# Autodesk Inventor assembly: RightSidePanelForCar
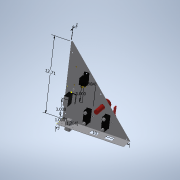
[picture p0: Inventor's stored thumbnail of the model, 180x180]
Saved by Autodesk Inventor 2021 (Build 250183000, 183)
## iProperties
Created: 2020-09-29
Part Number: RightSidePanelForCar
Document SubType Name: Assembly
Designer: Jonathan
Author: Jonathan
## Documents named in this file (9)
- D:\Scool\ECE 491\FullCarV2.2-20201122T225417Z-001\FullCarV2.2\SidePanels\RightSidePanelForCar.iam
- D:\Scool\ECE 491\Side_panels_11_1\RightSidePanel2020.ipt
- D:\Scool\ECE 491\FullCarV2.2-20201122T225417Z-001\FullCarV2.2\SidePanels\estop.ipt
- D:\Scool\ECE 491\FullCarV2.2-20201122T225417Z-001\FullCarV2.2\SidePanels\imdreset.ipt
- D:\Scool\ECE 491\FullCarV2.2-20201122T225417Z-001\FullCarV2.2\SidePanels\SSOK.ipt
- D:\Scool\ECE 491\FullCarV2.2-20201122T225417Z-001\FullCarV2.2\SidePanels\MRESET.iam
- D:\Scool\ECE 491\FullCarV2.2-20201122T225417Z-001\FullCarV2.2\SidePanels\DT_Flange_1.ipt
- D:\Scool\ECE 491\bosch-automotive-relay-0332209150-1.snapshot.3\Bosch 0 332 209 150.ipt
- D:\Scool\ECE 491\FullCarV2.2-20201122T225417Z-001\FullCarV2.2\SidePanels\9600K130_SBR RUBBER PUSH-IN GROMMET.ipt
## Components (9 placed, 8 different names)
1. RightSidePanel2020:1 — Mate:1, Mate:2, Mate:3, Mate:4, Mate:5, Mate:6, Mate:7, Mate:8, Mate:9, Mate:10, Mate:11, Mate:12, Mate:13, Insert:1, Mate:15, Mate:16
2. estop:1 — Mate:1, Mate:2
3. imdreset:1 — Mate:5, Mate:13
4. SSOK:1 — Mate:3, Mate:4, Mate:12
5. MRESET:1 [sub-assembly] — Mate:9, Mate:10, Mate:11
6. MRESET:2 [sub-assembly] — Mate:6, Mate:7, Mate:8
7. DT_Flange_1:1 — Mate:15
8. Bosch 0 332 209 150:1 — Mate:16
9. 9600K130_SBR RUBBER PUSH-IN GROMMET:1 — Insert:1
## Relationships (16: Mate 15, Insert 1)
- Mate:1: RightSidePanel2020:1 ↔ estop:1
- Mate:2: RightSidePanel2020:1 ↔ estop:1
- Mate:3: RightSidePanel2020:1 ↔ SSOK:1
- Mate:4: RightSidePanel2020:1 ↔ SSOK:1
- Mate:5: RightSidePanel2020:1 ↔ imdreset:1
- Mate:6: RightSidePanel2020:1 ↔ MRESET:2
- Mate:7: RightSidePanel2020:1 ↔ MRESET:2
- Mate:8: RightSidePanel2020:1 ↔ MRESET:2
- Mate:9: RightSidePanel2020:1 ↔ MRESET:1
- Mate:10: RightSidePanel2020:1 ↔ MRESET:1
- Mate:11: RightSidePanel2020:1 ↔ MRESET:1
- Mate:12: RightSidePanel2020:1 ↔ SSOK:1
- Mate:13: RightSidePanel2020:1 ↔ imdreset:1
- Insert:1: RightSidePanel2020:1 ↔ 9600K130_SBR RUBBER PUSH-IN GROMMET:1
- Mate:15: RightSidePanel2020:1 ↔ DT_Flange_1:1
- Mate:16: RightSidePanel2020:1 ↔ Bosch 0 332 209 150:1
